# Autodesk Inventor assembly: Cylinder Assembly
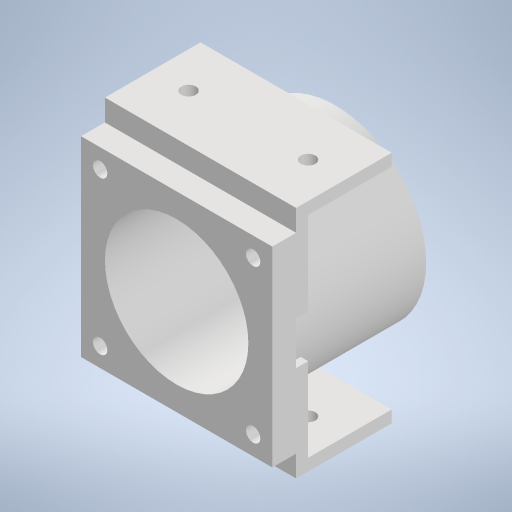
[picture p0: Inventor's stored thumbnail of the model, 512x512]
Saved by Autodesk Inventor 2023 (Build 270158000, 158)
## iProperties
Created: 2022-12-22
Part Number: Cylinder Assembly
Document SubType Name: Assembly
Designer: tgr41
Author: tgr41
## Documents named in this file (3)
- C:\Users\tgr41\OneDrive\Documents\Repositories\3D-Prints\Steam Engine 2 Inch V3\Cylinder Assembly.iam
- C:\Users\tgr41\OneDrive\Documents\Repositories\Steam-Engine\2 Inch V3\Cylinder Bracket.ipt
- C:\Users\tgr41\OneDrive\Documents\Repositories\Steam-Engine\2 Inch V3\Cylinders.ipt
## Components (3 placed, 2 different names)
1. Cylinder Bracket:1 — Mate:1, Mate:2, Mate:3
2. Cylinder Bracket:2 — Mate:4, Mate:5, Mate:6
3. Cylinders:1 — Mate:1, Mate:2, Mate:3, Mate:4, Mate:5, Mate:6
## Relationships (6: Mate 6)
- Mate:1: Cylinder Bracket:1 ↔ Cylinders:1
- Mate:2: Cylinder Bracket:1 ↔ Cylinders:1
- Mate:3: Cylinder Bracket:1 ↔ Cylinders:1
- Mate:4: Cylinder Bracket:2 ↔ Cylinders:1
- Mate:5: Cylinder Bracket:2 ↔ Cylinders:1
- Mate:6: Cylinder Bracket:2 ↔ Cylinders:1
